# Autodesk Inventor assembly: The Real Chassis
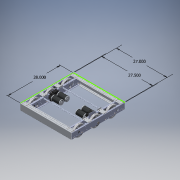
[picture p0: Inventor's stored thumbnail of the model, 180x180]
Saved by Autodesk Inventor 2018 (Build 220112000, 112)
## iProperties
Created: 2015-12-07
Part Number: The Real Chassis
Description: STEP AP214
Document SubType Name: Assembly
Designer: 20dbrownell
Sending System: SolidWorks 2014
Preprocessor: SwSTEP 2.0
Title: AM14U3 Square REV1-1.STEP
Revision Number: ANY
## Documents named in this file (3)
- C:\Users\20dbrownell\Documents\GitHub\RobotDesigns2018\The Real Chassis.iam
- C:\Users\20dbrownell\Downloads\AM14U3 Square Half.iam
- H:\Robotics\am-0255+2.5inch+CIM+Motor.ipt
## Components (6 placed, 3 different names)
1. AM14U3 Square Half_1 [sub-assembly] — Mate:1, Mate:2, Mate:5, Mate:6
2. AM14U3 Square Half_2 [sub-assembly] — Mate:3, Mate:4, Mate:7, Mate:8
3. am-0255+2.5inch+CIM+Motor:1 — Mate:4, Mate:7
4. am-0255+2.5inch+CIM+Motor:2 — Mate:3, Mate:8
5. am-0255+2.5inch+CIM+Motor:3 — Mate:2, Mate:6
6. am-0255+2.5inch+CIM+Motor:4 — Mate:1, Mate:5
## Relationships (8: Mate 8)
- Mate:1: AM14U3 Square Half_1 ↔ am-0255+2.5inch+CIM+Motor:4
- Mate:2: AM14U3 Square Half_1 ↔ am-0255+2.5inch+CIM+Motor:3
- Mate:3: AM14U3 Square Half_2 ↔ am-0255+2.5inch+CIM+Motor:2
- Mate:4: AM14U3 Square Half_2 ↔ am-0255+2.5inch+CIM+Motor:1
- Mate:5: AM14U3 Square Half_1 ↔ am-0255+2.5inch+CIM+Motor:4
- Mate:6: AM14U3 Square Half_1 ↔ am-0255+2.5inch+CIM+Motor:3
- Mate:7: AM14U3 Square Half_2 ↔ am-0255+2.5inch+CIM+Motor:1
- Mate:8: AM14U3 Square Half_2 ↔ am-0255+2.5inch+CIM+Motor:2
